# Autodesk Inventor assembly: Link3
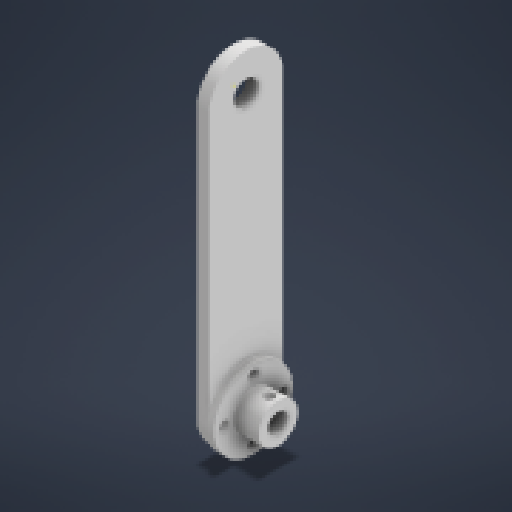
[picture p0: Inventor's stored thumbnail of the model, 512x512]
Saved by Autodesk Inventor 2023 (Build 270158000, 158)
## iProperties
Created: 2023-09-10
Part Number: Link3
Document SubType Name: Assembly
Designer: philo
Author: philo
## Documents named in this file (3)
- C:\Users\philo\OneDrive\Desktop\HK1-2024\TT ROBOT\02_3D_design_new\Link3.iam
- C:\Users\philo\OneDrive\Desktop\HK1-2024\TT ROBOT\02_3D_design_new\Link3Do.ipt
- C:\Users\philo\OneDrive\Desktop\HK1-2024\TT ROBOT\02_3D_design_new\trudong15mm.ipt
## Components (3 placed, 2 different names)
1. Link3Do:1 — Angle:1, Mate:3, Mate:4, Mate:5, Mate:6, Mate:7
2. Link3Do:2 — Mate:3, Mate:4, Mate:5
3. trudong15mm:1 — Mate:6, Mate:7
## Relationships (6: Mate 5, Angle 1)
- Angle:1 (0 deg): Link3Do:1
- Mate:3: Link3Do:1 ↔ Link3Do:2
- Mate:4: Link3Do:1 ↔ Link3Do:2
- Mate:5 (18 mm): Link3Do:1 ↔ Link3Do:2
- Mate:6: Link3Do:1 ↔ trudong15mm:1
- Mate:7: Link3Do:1 ↔ trudong15mm:1
